# Autodesk Inventor assembly: Catapult Launcher
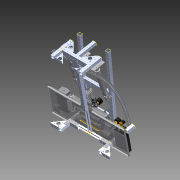
[picture p0: Inventor's stored thumbnail of the model, 180x180]
Saved by Autodesk Inventor 2014 SP1 (Build 180222100, 222)
## iProperties
Created: 2014-01-17
Part Number: Catapult Launcher
Document SubType Name: Assembly
Designer: Andrew Toennies
Mass: 5501.43 g
Surface Area: 13469.8 cm^2
Volume: 1150.51 cm^3
Density: 4.78173 g/cm^3
Author: Andrew Toennies
## Documents named in this file (38)
- C:\Users\Arpan\Documents\GitHub\2014buildCAD\New Shooter\Catapult Launcher.iam
- C:\Users\Arpan\Documents\GitHub\2014buildCAD\New Shooter\Vex Pro Side Bearing Gusset - OUT OF STOCK 1192014.ipt
- C:\Users\Arpan\Documents\GitHub\2014buildCAD\New Shooter\Vex Pro Corner Gusset - IN STOCK 1192014.ipt
- C:\Users\Arpan\Documents\GitHub\2014buildCAD\New Shooter\Bearing ID 0.500 Hex OD 1.125.ipt
- C:\Users\Arpan\Documents\GitHub\2014buildCAD\New Shooter\Shaft (Steel 0.500 Hex).ipt
- C:\Users\Arpan\Documents\GitHub\2014buildCAD\New Shooter\1.5 in bore 6 in stroke cylinder - BIMBA\176-DP(D-229)(F,D-231-1).iam
- C:\Users\Arpan\Documents\GitHub\2014buildCAD\New Shooter\Aluminum Plate (0.125).ipt
- C:\Users\Arpan\Documents\GitHub\2014buildCAD\New Shooter\1.5 in bore 6 in stroke cylinder - BIMBA\D-14826.ipt
- C:\Users\Arpan\Documents\GitHub\2014buildCAD\New Shooter\1.5 in bore 6 in stroke cylinder - BIMBA\D-9969.ipt
- C:\Users\Arpan\Documents\GitHub\2014buildCAD\New Shooter\Vex Pro End Bearing Mount - IN STOCK 1192014.ipt
- C:\Users\Arpan\Documents\GitHub\2014buildCAD\New Shooter\Vex Pro 1x1 rectangular tubing 13 in length.ipt
- C:\Users\Arpan\Documents\GitHub\2014buildCAD\New Shooter\Vex Pro 1x1 rectangular tubing 25 in length.ipt
- C:\Users\Arpan\Documents\GitHub\2014buildCAD\New Shooter\0.5625 in bore 2 in stroke compact cylinder - BIMBA\FO-022.iam
- C:\Users\Arpan\Documents\GitHub\2014buildCAD\New Shooter\Hex Shaft Collar 1-2 in (7552K500).ipt
- C:\Users\Arpan\Documents\GitHub\2014buildCAD\New Shooter\#8 1 in length standoff 93330A459.ipt
- C:\Users\Arpan\Documents\GitHub\2014buildCAD\New Shooter\Ramp.ipt
- C:\Users\Arpan\Documents\GitHub\2014buildCAD\New folder (2)\Pneumatics_Clippard_AVT-32-16.iam
- C:\Users\Arpan\Documents\GitHub\2014buildCAD\New Shooter\Vex Pro T gusset - OUT OF STOCK 1192014.ipt
- C:\Users\Arpan\Documents\GitHub\2014buildCAD\New Shooter\#8 0.250 in length spacer 92510A462.ipt
- C:\Users\Arpan\Documents\GitHub\2014buildCAD\New Shooter\#8 0.625 in length spacer 92510A466.ipt
- C:\Users\Arpan\Documents\GitHub\2014buildCAD\New Shooter\Vex Pro 1x1 rectangular tubing 12 in length.ipt
- C:\Users\Arpan\Documents\GitHub\2014buildCAD\New Shooter\Vex Pro 1x1 rectangular tubing 24.5 in length.ipt
- C:\Users\Arpan\Documents\GitHub\2014buildCAD\New Shooter\Vex Pro 1x1 rectangular tubing 7 in length.ipt
- C:\Users\Arpan\Documents\GitHub\2014buildCAD\New Shooter\Vex Pro 1x1 rectangular tubing 9 in length.ipt
- C:\Users\Arpan\Documents\GitHub\2014buildCAD\New Shooter\Vex Pro 1x1 rectangular tubing 6.125 in length.ipt
- C:\Users\Arpan\Documents\GitHub\2014buildCAD\New Shooter\Spacer (0.630 in ID 1 in OD) aluminum.ipt
- C:\Users\Arpan\Documents\GitHub\2014buildCAD\big air tank\Pneumatics_Clippard_AVT-32-32.iam
- C:\Users\Arpan\Documents\GitHub\2014buildCAD\pneumatics board\pneumatics thing 2.iam
- C:\Users\Arpan\Documents\GitHub\2014buildCAD\New Shooter\Manifold and Valves\Manifold.iam
- C:\Users\Arpan\Documents\GitHub\2014buildCAD\pneumatics board\pneumatic thing 1.iam
- C:\Users\Arpan\Documents\GitHub\2014buildCAD\electrical\CS_Converter_CLL25-24S05.ipt
- C:\Users\Arpan\Documents\GitHub\2014buildCAD\electrical\CS_WirelessBridge_DAP1522.ipt
- C:\Users\Arpan\Documents\GitHub\2014buildCAD\New Shooter\Pneumatics Board.ipt
- C:\Users\Arpan\Documents\GitHub\2014buildCAD\New Shooter\Aluminum Angle 2.ipt
- C:\Users\Arpan\Documents\GitHub\2014buildCAD\New Shooter\Aluminum Angle 1 Left.ipt
- C:\Users\Arpan\Documents\GitHub\2014buildCAD\New Shooter\Aluminum Angle 1 Right.ipt
- C:\Users\Arpan\Documents\GitHub\2014buildCAD\New Shooter\Aluminum Angle 3 Left.ipt
- C:\Users\Arpan\Documents\GitHub\2014buildCAD\New Shooter\Aluminum Angle 3 Right.ipt
## Components (98 placed, 37 different names)
1. Vex Pro T gusset - OUT OF STOCK 1192014:2 — Mate:376, Flush:71, Flush:72
2. Vex Pro T gusset - OUT OF STOCK 1192014:1 — Mate:375, Flush:69, Flush:70
3. #8 1 in length standoff 93330A459:12 — Mate:342, Mate:343
4. #8 1 in length standoff 93330A459:11 — Mate:340, Mate:341
5. #8 1 in length standoff 93330A459:10 — Mate:338, Mate:339
6. #8 1 in length standoff 93330A459:9 — Mate:336, Mate:337
7. #8 1 in length standoff 93330A459:6 — Mate:325, Mate:326
8. #8 1 in length standoff 93330A459:1 — Mate:319, Mate:320
9. #8 1 in length standoff 93330A459:2 — Mate:321, Mate:322
10. #8 1 in length standoff 93330A459:5 — Mate:323, Mate:324
11. Vex Pro 1x1 rectangular tubing 12 in length:1 — Flush:1, Flush:2, Mate:8, Mate:11, Mate:195, Flush:32, Flush:33, Flush:34, Flush:35, Mate:278, Flush:51, Mate:352, Mate:376, Flush:71, Mate:380, Mate:381, Mate:390, Flush:77, Flush:78, Mate:403, Mate:405
12. Vex Pro 1x1 rectangular tubing 12 in length:2 — Flush:1, Flush:2, Mate:3, Mate:5, Mate:123, Mate:188, Mate:195, Flush:25, Flush:28, Flush:29, Flush:30, Flush:31, Mate:355, Mate:375, Flush:69, Mate:378, Mate:389, Flush:75, Flush:76
13. Vex Pro Side Bearing Gusset - OUT OF STOCK 1192014:1 — Mate:3, Mate:26, Mate:27, Flush:28, Flush:29, Mate:319, Mate:320, Mate:322, Mate:324, Mate:326
14. Vex Pro Side Bearing Gusset - OUT OF STOCK 1192014:2 — Mate:5, Mate:28, Mate:29, Flush:30, Flush:31, Mate:321, Mate:323, Mate:325
15. Vex Pro Side Bearing Gusset - OUT OF STOCK 1192014:3 — Mate:11, Mate:32, Mate:33, Flush:32, Flush:33, Mate:337, Mate:338, Mate:339, Mate:340, Mate:342, Mate:343
16. Vex Pro Side Bearing Gusset - OUT OF STOCK 1192014:4 — Mate:8, Mate:30, Mate:31, Flush:34, Flush:35, Mate:336, Mate:341
17. Vex Pro Corner Gusset - IN STOCK 1192014:2 — Mate:389, Flush:75, Flush:76
18. Vex Pro Corner Gusset - IN STOCK 1192014:4 — Mate:390, Flush:77, Flush:78
19. Bearing ID 0.500 Hex OD 1.125:1 — Mate:28, Mate:29, Flush:3, Flush:5, Mate:306
20. Bearing ID 0.500 Hex OD 1.125:2 — Mate:26, Mate:27, Flush:3, Mate:34, Mate:35, Mate:303
21. Bearing ID 0.500 Hex OD 1.125:3 — Mate:30, Mate:31, Flush:4, Mate:318
22. Bearing ID 0.500 Hex OD 1.125:4 — Mate:32, Mate:33, Flush:4, Flush:5, Mate:69, Mate:315
23. Pneumatics_Clippard_AVT-32-16:1 [sub-assembly] — Tangent:8, Flush:94, Tangent:11, Tangent:12
24. Pneumatics_Clippard_AVT-32-16:2 [sub-assembly] — Tangent:10, Flush:94, Tangent:11, Tangent:13, Flush:101
25. Pneumatics_Clippard_AVT-32-32:1 [sub-assembly] — Mate:403, Tangent:2, Flush:87, Tangent:9, Tangent:12
26. Pneumatics_Clippard_AVT-32-32:2 [sub-assembly] — Flush:87, Tangent:7, Tangent:13, Flush:101
27. Manifold:1 [sub-assembly] — Mate:406, Flush:97, Flush:98
28. pneumatic thing 1:1 [sub-assembly] — Mate:408, Flush:92, Flush:93
29. CS_Converter_CLL25-24S05:1 — Mate:410, Mate:414, Mate:415
30. CS_WirelessBridge_DAP1522:1 — Mate:409, Flush:90, Flush:91
31. Pneumatics Board:1 — Mate:404, Mate:405, Flush:89, Mate:406, Mate:408, Mate:409, Mate:410, Flush:90, Flush:91, Flush:92, Flush:93, Tangent:7, Tangent:8, Tangent:9, Tangent:10, Mate:413, Flush:97, Mate:414, Mate:415, Flush:98, Flush:99, Flush:100, Mate:418, Flush:102, Mate:419, Mate:420, Flush:103, Mate:421, Flush:104, Mate:422, Mate:423, Mate:424, Mate:425, Flush:105, Mate:426, Flush:106, Mate:428, Flush:107
32. pneumatics thing 2:2 [sub-assembly] — Mate:413, Flush:99, Flush:100
33. #8 1 in length standoff 93330A459:13 — Mate:350, Mate:351
34. #8 1 in length standoff 93330A459:14 — Mate:348, Mate:349
35. #8 1 in length standoff 93330A459:15 — Mate:346, Mate:347
36. #8 1 in length standoff 93330A459:16 — Mate:344, Mate:345
37. #8 1 in length standoff 93330A459:3 — Mate:327, Mate:328
38. #8 1 in length standoff 93330A459:4 — Mate:329, Mate:330
39. #8 1 in length standoff 93330A459:7 — Mate:334, Mate:335
40. #8 1 in length standoff 93330A459:8 — Mate:332, Mate:333
41. Vex Pro Corner Gusset - IN STOCK 1192014:14 — Mate:250, Mate:251, Flush:45, Mate:271
42. Vex Pro Corner Gusset - IN STOCK 1192014:13 — Mate:252, Mate:253, Flush:46
43. Vex Pro Corner Gusset - IN STOCK 1192014:12 — Mate:248, Mate:249, Flush:44
44. Vex Pro Corner Gusset - IN STOCK 1192014:11 — Mate:243, Flush:43, Mate:244
45. Vex Pro 1x1 rectangular tubing 9 in length:1 — Mate:191, Flush:42, Mate:250, Mate:253, Flush:46, Mate:267
46. Vex Pro 1x1 rectangular tubing 9 in length:2 — Flush:41, Mate:242, Mate:243, Flush:43, Mate:246, Mate:248, Flush:44
47. D-9969:1 — Mate:164, Mate:165, Mate:198, Flush:36, Mate:270, Mate:377
48. D-14826:1 — Mate:164, Mate:169, Mate:170, Flush:37, Mate:247
49. Vex Pro End Bearing Mount - IN STOCK 1192014:4 — Mate:229, Mate:230, Mate:231, Mate:232, Mate:246, Mate:345, Mate:346, Mate:348, Mate:349, Mate:350
50. Vex Pro End Bearing Mount - IN STOCK 1192014:3 — Mate:217, Mate:218, Mate:219, Mate:220, Mate:221, Mate:327, Mate:328, Mate:330, Mate:333, Mate:335
51. Vex Pro End Bearing Mount - IN STOCK 1192014:2 — Mate:233, Mate:234, Mate:235, Mate:236, Mate:245, Mate:344, Mate:347, Mate:351
52. Vex Pro End Bearing Mount - IN STOCK 1192014:1 — Mate:222, Mate:223, Mate:224, Mate:225, Mate:226, Mate:329, Mate:332, Mate:334
53. Vex Pro 1x1 rectangular tubing 24.5 in length:2 — Mate:198, Mate:229, Mate:230, Mate:231, Mate:233, Mate:234, Mate:235, Flush:27, Flush:36, Flush:41, Mate:242, Mate:244, Mate:251, Flush:45, Mate:267, Mate:270, Mate:271
54. Vex Pro 1x1 rectangular tubing 24.5 in length:1 — Mate:188, Mate:191, Mate:212, Mate:219, Mate:220, Mate:221, Mate:224, Mate:225, Mate:226, Flush:26, Flush:37, Flush:42, Mate:247, Mate:249, Mate:252
55. Bearing ID 0.500 Hex OD 1.125:5 — Mate:80, Mate:222, Mate:223, Mate:228, Mate:309
56. Bearing ID 0.500 Hex OD 1.125:6 — Mate:80, Mate:217, Mate:218, Mate:227
57. Bearing ID 0.500 Hex OD 1.125:7 — Mate:68, Mate:69, Mate:236, Mate:245, Mate:397
58. Bearing ID 0.500 Hex OD 1.125:8 — Mate:68, Mate:232, Mate:312
59. Vex Pro T gusset - OUT OF STOCK 1192014:3 — Mate:388, Flush:73, Flush:74
60. Aluminum Plate (0.125):1 — Mate:153, Mate:159, Mate:434, Mate:435, Mate:436, Mate:437
61. Aluminum Plate (0.125):2 — Mate:156, Mate:160, Mate:430, Mate:431, Mate:432, Mate:433
62. Vex Pro 1x1 rectangular tubing 7 in length:2 — Flush:19, Mate:159, Flush:27, Mate:276, Mate:359, Mate:385, Mate:391, Flush:79, Flush:80, Mate:430, Mate:431
63. Vex Pro 1x1 rectangular tubing 7 in length:1 — Mate:123, Flush:19, Mate:160, Mate:212, Flush:26, Mate:272, Flush:48, Mate:273, Mate:275, Mate:360, Mate:387, Mate:392, Flush:81, Flush:82, Mate:434, Mate:435
64. Vex Pro Corner Gusset - IN STOCK 1192014:8 — Mate:392, Flush:81, Flush:82
65. Vex Pro Corner Gusset - IN STOCK 1192014:6 — Mate:391, Flush:79, Flush:80
66. Vex Pro 1x1 rectangular tubing 9 in length:3 — Mate:272, Flush:48, Mate:274, Flush:49, Mate:277, Flush:50, Mate:290, Mate:291, Mate:293, Flush:57, Mate:369, Flush:66
67. Vex Pro Corner Gusset - IN STOCK 1192014:15 — Mate:273, Mate:274, Flush:49, Mate:275
68. Vex Pro Corner Gusset - IN STOCK 1192014:16 — Mate:276, Mate:277, Flush:50
69. Vex Pro 1x1 rectangular tubing 13 in length:1 — Mate:278, Flush:51, Mate:284, Flush:55, Flush:70, Flush:72, Mate:388, Flush:73, Tangent:2, Mate:404, Flush:89
70. Vex Pro 1x1 rectangular tubing 25 in length:1 — Mate:284, Flush:55, Mate:285, Mate:289, Flush:56, Mate:292, Mate:300, Flush:67, Flush:74, Mate:416, Mate:417
71. FO-022:1 [sub-assembly] — Mate:285, Mate:416, Mate:417
72. Vex Pro Corner Gusset - IN STOCK 1192014:17 — Mate:289, Mate:290, Flush:56, Mate:291
73. Vex Pro Corner Gusset - IN STOCK 1192014:18 — Mate:292, Mate:293, Flush:57
74. Vex Pro 1x1 rectangular tubing 6.125 in length:1 — Mate:369, Flush:66, Mate:370, Flush:68
75. Vex Pro Corner Gusset - IN STOCK 1192014:21 — Mate:300, Mate:370, Flush:67, Flush:68
76. #8 0.250 in length spacer 92510A462:1 — Mate:380, Mate:381, Mate:382
77. #8 0.250 in length spacer 92510A462:2 — Mate:378, Mate:379, Mate:383
78. #8 0.625 in length spacer 92510A466:1 — Mate:384, Mate:385
79. #8 0.625 in length spacer 92510A466:2 — Mate:386, Mate:387
80. Ramp:1 — Mate:355, Mate:360, Mate:379, Mate:383, Mate:386
81. Ramp:2 — Mate:352, Mate:359, Mate:382, Mate:384
82. Aluminum Angle 2:1 — Mate:418, Flush:102, Mate:419, Mate:429
83. Aluminum Angle 2:2 — Mate:420, Flush:103, Mate:421, Mate:427
84. Aluminum Angle 1 Left:1 — Flush:104, Mate:422, Mate:423
85. Aluminum Angle 1 Right:1 — Mate:424, Mate:425, Flush:105
86. Aluminum Angle 3 Left:1 — Mate:426, Flush:106, Mate:427
87. Aluminum Angle 3 Right:1 — Mate:428, Mate:429, Flush:107
88. Spacer (0.630 in ID 1 in OD) aluminum:1 — Mate:399, Mate:400
89. Spacer (0.630 in ID 1 in OD) aluminum:2 — Mate:397, Mate:398
90. Shaft (Steel 0.500 Hex):1 — Mate:34, Mate:35, Flush:25, Mate:227, Mate:228, Mate:301, Mate:302, Mate:304, Mate:305, Mate:307, Mate:308, Mate:310, Mate:311, Mate:313, Mate:314, Mate:316, Mate:317
91. Hex Shaft Collar 1-2 in (7552K500):1 — Mate:301, Mate:302, Mate:303
92. Hex Shaft Collar 1-2 in (7552K500):2 — Mate:307, Mate:308, Mate:309
93. Hex Shaft Collar 1-2 in (7552K500):3 — Mate:304, Mate:305, Mate:306, Mate:399, Mate:400
94. Hex Shaft Collar 1-2 in (7552K500):4 — Mate:310, Mate:311, Mate:312
95. Hex Shaft Collar 1-2 in (7552K500):5 — Mate:313, Mate:314, Mate:315, Mate:398
96. Hex Shaft Collar 1-2 in (7552K500):6 — Mate:316, Mate:317, Mate:318
97. 176-DP(D-229)(F,D-231-1):1 [sub-assembly] — Mate:153, Mate:165, Mate:171, Mate:377, Mate:432, Mate:433
98. 176-DP(D-229)(F,D-231-1):2 [sub-assembly] — Mate:156, Mate:169, Mate:170, Mate:171, Mate:436, Mate:437
## Relationships (267: Mate 192, Flush 67, Tangent 8)
- Flush:1: Vex Pro 1x1 rectangular tubing 12 in length:1 ↔ Vex Pro 1x1 rectangular tubing 12 in length:2
- Flush:2: Vex Pro 1x1 rectangular tubing 12 in length:1 ↔ Vex Pro 1x1 rectangular tubing 12 in length:2
- Mate:3: Vex Pro 1x1 rectangular tubing 12 in length:2 ↔ Vex Pro Side Bearing Gusset - OUT OF STOCK 1192014:1
- Mate:5: Vex Pro 1x1 rectangular tubing 12 in length:2 ↔ Vex Pro Side Bearing Gusset - OUT OF STOCK 1192014:2
- Mate:8: Vex Pro 1x1 rectangular tubing 12 in length:1 ↔ Vex Pro Side Bearing Gusset - OUT OF STOCK 1192014:4
- Mate:11: Vex Pro 1x1 rectangular tubing 12 in length:1 ↔ Vex Pro Side Bearing Gusset - OUT OF STOCK 1192014:3
- Mate:26: Vex Pro Side Bearing Gusset - OUT OF STOCK 1192014:1 ↔ Bearing ID 0.500 Hex OD 1.125:2
- Mate:27: Vex Pro Side Bearing Gusset - OUT OF STOCK 1192014:1 ↔ Bearing ID 0.500 Hex OD 1.125:2
- Mate:28: Vex Pro Side Bearing Gusset - OUT OF STOCK 1192014:2 ↔ Bearing ID 0.500 Hex OD 1.125:1
- Mate:29: Vex Pro Side Bearing Gusset - OUT OF STOCK 1192014:2 ↔ Bearing ID 0.500 Hex OD 1.125:1
- Flush:3: Bearing ID 0.500 Hex OD 1.125:1 ↔ Bearing ID 0.500 Hex OD 1.125:2
- Mate:30: Vex Pro Side Bearing Gusset - OUT OF STOCK 1192014:4 ↔ Bearing ID 0.500 Hex OD 1.125:3
- Mate:31: Vex Pro Side Bearing Gusset - OUT OF STOCK 1192014:4 ↔ Bearing ID 0.500 Hex OD 1.125:3
- Mate:32: Vex Pro Side Bearing Gusset - OUT OF STOCK 1192014:3 ↔ Bearing ID 0.500 Hex OD 1.125:4
- Mate:33: Vex Pro Side Bearing Gusset - OUT OF STOCK 1192014:3 ↔ Bearing ID 0.500 Hex OD 1.125:4
- Flush:4: Bearing ID 0.500 Hex OD 1.125:3 ↔ Bearing ID 0.500 Hex OD 1.125:4
- Flush:5: Bearing ID 0.500 Hex OD 1.125:1 ↔ Bearing ID 0.500 Hex OD 1.125:4
- Mate:34: Bearing ID 0.500 Hex OD 1.125:2 ↔ Shaft (Steel 0.500 Hex):1
- Mate:35: Bearing ID 0.500 Hex OD 1.125:2 ↔ Shaft (Steel 0.500 Hex):1
- Mate:68: Bearing ID 0.500 Hex OD 1.125:7 ↔ Bearing ID 0.500 Hex OD 1.125:8
- Mate:69: Bearing ID 0.500 Hex OD 1.125:4 ↔ Bearing ID 0.500 Hex OD 1.125:7
- Mate:80: Bearing ID 0.500 Hex OD 1.125:5 ↔ Bearing ID 0.500 Hex OD 1.125:6
- Mate:123 (-685.8 mm): Vex Pro 1x1 rectangular tubing 12 in length:2 ↔ Vex Pro 1x1 rectangular tubing 7 in length:1
- Flush:19: Vex Pro 1x1 rectangular tubing 7 in length:2 ↔ Vex Pro 1x1 rectangular tubing 7 in length:1
- Mate:153: Aluminum Plate (0.125):1 ↔ 176-DP(D-229)(F,D-231-1):1
- Mate:156: Aluminum Plate (0.125):2 ↔ 176-DP(D-229)(F,D-231-1):2
- Mate:159: Aluminum Plate (0.125):1 ↔ Vex Pro 1x1 rectangular tubing 7 in length:2
- Mate:160: Aluminum Plate (0.125):2 ↔ Vex Pro 1x1 rectangular tubing 7 in length:1
- Mate:164: D-9969:1 ↔ D-14826:1
- Mate:165: D-9969:1 ↔ 176-DP(D-229)(F,D-231-1):1
- Mate:169: D-14826:1 ↔ 176-DP(D-229)(F,D-231-1):2
- Mate:170: D-14826:1 ↔ 176-DP(D-229)(F,D-231-1):2
- Mate:171: 176-DP(D-229)(F,D-231-1):1 ↔ 176-DP(D-229)(F,D-231-1):2
- Mate:188 (25.4 mm): Vex Pro 1x1 rectangular tubing 12 in length:2 ↔ Vex Pro 1x1 rectangular tubing 24.5 in length:1
- Mate:191: Vex Pro 1x1 rectangular tubing 9 in length:1 ↔ Vex Pro 1x1 rectangular tubing 24.5 in length:1
- Mate:195 (330.2 mm): Vex Pro 1x1 rectangular tubing 12 in length:1 ↔ Vex Pro 1x1 rectangular tubing 12 in length:2
- Flush:25 (-25.4 mm): Vex Pro 1x1 rectangular tubing 12 in length:2 ↔ Shaft (Steel 0.500 Hex):1
- Mate:198: D-9969:1 ↔ Vex Pro 1x1 rectangular tubing 24.5 in length:2
- Mate:212: Vex Pro 1x1 rectangular tubing 24.5 in length:1 ↔ Vex Pro 1x1 rectangular tubing 7 in length:1
- Mate:217: Vex Pro End Bearing Mount - IN STOCK 1192014:3 ↔ Bearing ID 0.500 Hex OD 1.125:6
- Mate:218: Vex Pro End Bearing Mount - IN STOCK 1192014:3 ↔ Bearing ID 0.500 Hex OD 1.125:6
- Mate:219: Vex Pro End Bearing Mount - IN STOCK 1192014:3 ↔ Vex Pro 1x1 rectangular tubing 24.5 in length:1
- Mate:220: Vex Pro End Bearing Mount - IN STOCK 1192014:3 ↔ Vex Pro 1x1 rectangular tubing 24.5 in length:1
- Mate:221: Vex Pro End Bearing Mount - IN STOCK 1192014:3 ↔ Vex Pro 1x1 rectangular tubing 24.5 in length:1
- Mate:222: Vex Pro End Bearing Mount - IN STOCK 1192014:1 ↔ Bearing ID 0.500 Hex OD 1.125:5
- Mate:223: Vex Pro End Bearing Mount - IN STOCK 1192014:1 ↔ Bearing ID 0.500 Hex OD 1.125:5
- Mate:224: Vex Pro End Bearing Mount - IN STOCK 1192014:1 ↔ Vex Pro 1x1 rectangular tubing 24.5 in length:1
- Mate:225: Vex Pro End Bearing Mount - IN STOCK 1192014:1 ↔ Vex Pro 1x1 rectangular tubing 24.5 in length:1
- Mate:226: Vex Pro End Bearing Mount - IN STOCK 1192014:1 ↔ Vex Pro 1x1 rectangular tubing 24.5 in length:1
- Mate:227: Bearing ID 0.500 Hex OD 1.125:6 ↔ Shaft (Steel 0.500 Hex):1
- Mate:228: Bearing ID 0.500 Hex OD 1.125:5 ↔ Shaft (Steel 0.500 Hex):1
- Mate:229: Vex Pro End Bearing Mount - IN STOCK 1192014:4 ↔ Vex Pro 1x1 rectangular tubing 24.5 in length:2
- Mate:230: Vex Pro End Bearing Mount - IN STOCK 1192014:4 ↔ Vex Pro 1x1 rectangular tubing 24.5 in length:2
- Mate:231: Vex Pro End Bearing Mount - IN STOCK 1192014:4 ↔ Vex Pro 1x1 rectangular tubing 24.5 in length:2
- Mate:232: Vex Pro End Bearing Mount - IN STOCK 1192014:4 ↔ Bearing ID 0.500 Hex OD 1.125:8
- Mate:233: Vex Pro End Bearing Mount - IN STOCK 1192014:2 ↔ Vex Pro 1x1 rectangular tubing 24.5 in length:2
- Mate:234: Vex Pro End Bearing Mount - IN STOCK 1192014:2 ↔ Vex Pro 1x1 rectangular tubing 24.5 in length:2
- Mate:235: Vex Pro End Bearing Mount - IN STOCK 1192014:2 ↔ Vex Pro 1x1 rectangular tubing 24.5 in length:2
- Mate:236: Vex Pro End Bearing Mount - IN STOCK 1192014:2 ↔ Bearing ID 0.500 Hex OD 1.125:7
- Flush:26: Vex Pro 1x1 rectangular tubing 24.5 in length:1 ↔ Vex Pro 1x1 rectangular tubing 7 in length:1
- Flush:27: Vex Pro 1x1 rectangular tubing 24.5 in length:2 ↔ Vex Pro 1x1 rectangular tubing 7 in length:2
- Flush:28: Vex Pro 1x1 rectangular tubing 12 in length:2 ↔ Vex Pro Side Bearing Gusset - OUT OF STOCK 1192014:1
- Flush:29 (82.55 mm): Vex Pro 1x1 rectangular tubing 12 in length:2 ↔ Vex Pro Side Bearing Gusset - OUT OF STOCK 1192014:1
- Flush:30: Vex Pro 1x1 rectangular tubing 12 in length:2 ↔ Vex Pro Side Bearing Gusset - OUT OF STOCK 1192014:2
- Flush:31 (-82.55 mm): Vex Pro 1x1 rectangular tubing 12 in length:2 ↔ Vex Pro Side Bearing Gusset - OUT OF STOCK 1192014:2
- Flush:32: Vex Pro 1x1 rectangular tubing 12 in length:1 ↔ Vex Pro Side Bearing Gusset - OUT OF STOCK 1192014:3
- Flush:33 (82.55 mm): Vex Pro 1x1 rectangular tubing 12 in length:1 ↔ Vex Pro Side Bearing Gusset - OUT OF STOCK 1192014:3
- Flush:34: Vex Pro 1x1 rectangular tubing 12 in length:1 ↔ Vex Pro Side Bearing Gusset - OUT OF STOCK 1192014:4
- Flush:35 (-82.55 mm): Vex Pro 1x1 rectangular tubing 12 in length:1 ↔ Vex Pro Side Bearing Gusset - OUT OF STOCK 1192014:4
- Flush:36: D-9969:1 ↔ Vex Pro 1x1 rectangular tubing 24.5 in length:2
- Flush:37: D-14826:1 ↔ Vex Pro 1x1 rectangular tubing 24.5 in length:1
- Flush:41: Vex Pro 1x1 rectangular tubing 9 in length:2 ↔ Vex Pro 1x1 rectangular tubing 24.5 in length:2
- Mate:242: Vex Pro 1x1 rectangular tubing 9 in length:2 ↔ Vex Pro 1x1 rectangular tubing 24.5 in length:2
- Flush:42: Vex Pro 1x1 rectangular tubing 9 in length:1 ↔ Vex Pro 1x1 rectangular tubing 24.5 in length:1
- Mate:243: Vex Pro Corner Gusset - IN STOCK 1192014:11 ↔ Vex Pro 1x1 rectangular tubing 9 in length:2
- Flush:43: Vex Pro Corner Gusset - IN STOCK 1192014:11 ↔ Vex Pro 1x1 rectangular tubing 9 in length:2
- Mate:244: Vex Pro Corner Gusset - IN STOCK 1192014:11 ↔ Vex Pro 1x1 rectangular tubing 24.5 in length:2
- Mate:245: Vex Pro End Bearing Mount - IN STOCK 1192014:2 ↔ Bearing ID 0.500 Hex OD 1.125:7
- Mate:246 (6.35 mm): Vex Pro 1x1 rectangular tubing 9 in length:2 ↔ Vex Pro End Bearing Mount - IN STOCK 1192014:4
- Mate:247: D-14826:1 ↔ Vex Pro 1x1 rectangular tubing 24.5 in length:1
- Mate:248: Vex Pro Corner Gusset - IN STOCK 1192014:12 ↔ Vex Pro 1x1 rectangular tubing 9 in length:2
- Mate:249: Vex Pro Corner Gusset - IN STOCK 1192014:12 ↔ Vex Pro 1x1 rectangular tubing 24.5 in length:1
- Flush:44: Vex Pro Corner Gusset - IN STOCK 1192014:12 ↔ Vex Pro 1x1 rectangular tubing 9 in length:2
- Mate:250: Vex Pro Corner Gusset - IN STOCK 1192014:14 ↔ Vex Pro 1x1 rectangular tubing 9 in length:1
- Mate:251: Vex Pro Corner Gusset - IN STOCK 1192014:14 ↔ Vex Pro 1x1 rectangular tubing 24.5 in length:2
- Flush:45: Vex Pro Corner Gusset - IN STOCK 1192014:14 ↔ Vex Pro 1x1 rectangular tubing 24.5 in length:2
- Mate:252: Vex Pro Corner Gusset - IN STOCK 1192014:13 ↔ Vex Pro 1x1 rectangular tubing 24.5 in length:1
- Mate:253: Vex Pro Corner Gusset - IN STOCK 1192014:13 ↔ Vex Pro 1x1 rectangular tubing 9 in length:1
- Flush:46: Vex Pro Corner Gusset - IN STOCK 1192014:13 ↔ Vex Pro 1x1 rectangular tubing 9 in length:1
- Mate:267: Vex Pro 1x1 rectangular tubing 9 in length:1 ↔ Vex Pro 1x1 rectangular tubing 24.5 in length:2
- Mate:270: D-9969:1 ↔ Vex Pro 1x1 rectangular tubing 24.5 in length:2
- Mate:271: Vex Pro Corner Gusset - IN STOCK 1192014:14 ↔ Vex Pro 1x1 rectangular tubing 24.5 in length:2
- Mate:272: Vex Pro 1x1 rectangular tubing 7 in length:1 ↔ Vex Pro 1x1 rectangular tubing 9 in length:3
- Flush:48: Vex Pro 1x1 rectangular tubing 7 in length:1 ↔ Vex Pro 1x1 rectangular tubing 9 in length:3
- Mate:273: Vex Pro 1x1 rectangular tubing 7 in length:1 ↔ Vex Pro Corner Gusset - IN STOCK 1192014:15
- Mate:274: Vex Pro 1x1 rectangular tubing 9 in length:3 ↔ Vex Pro Corner Gusset - IN STOCK 1192014:15
- Flush:49: Vex Pro 1x1 rectangular tubing 9 in length:3 ↔ Vex Pro Corner Gusset - IN STOCK 1192014:15
- Mate:275: Vex Pro 1x1 rectangular tubing 7 in length:1 ↔ Vex Pro Corner Gusset - IN STOCK 1192014:15
- Mate:276: Vex Pro 1x1 rectangular tubing 7 in length:2 ↔ Vex Pro Corner Gusset - IN STOCK 1192014:16
- Mate:277: Vex Pro 1x1 rectangular tubing 9 in length:3 ↔ Vex Pro Corner Gusset - IN STOCK 1192014:16
- Flush:50: Vex Pro 1x1 rectangular tubing 9 in length:3 ↔ Vex Pro Corner Gusset - IN STOCK 1192014:16
- Mate:278: Vex Pro 1x1 rectangular tubing 12 in length:1 ↔ Vex Pro 1x1 rectangular tubing 13 in length:1
- Flush:51: Vex Pro 1x1 rectangular tubing 12 in length:1 ↔ Vex Pro 1x1 rectangular tubing 13 in length:1
- Mate:284: Vex Pro 1x1 rectangular tubing 13 in length:1 ↔ Vex Pro 1x1 rectangular tubing 25 in length:1
- Flush:55: Vex Pro 1x1 rectangular tubing 13 in length:1 ↔ Vex Pro 1x1 rectangular tubing 25 in length:1
- Mate:285: Vex Pro 1x1 rectangular tubing 25 in length:1 ↔ FO-022:1
- Mate:289: Vex Pro 1x1 rectangular tubing 25 in length:1 ↔ Vex Pro Corner Gusset - IN STOCK 1192014:17
- Mate:290: Vex Pro 1x1 rectangular tubing 9 in length:3 ↔ Vex Pro Corner Gusset - IN STOCK 1192014:17
- Flush:56: Vex Pro 1x1 rectangular tubing 25 in length:1 ↔ Vex Pro Corner Gusset - IN STOCK 1192014:17
- Mate:291: Vex Pro 1x1 rectangular tubing 9 in length:3 ↔ Vex Pro Corner Gusset - IN STOCK 1192014:17
- Mate:292: Vex Pro 1x1 rectangular tubing 25 in length:1 ↔ Vex Pro Corner Gusset - IN STOCK 1192014:18
- Mate:293: Vex Pro 1x1 rectangular tubing 9 in length:3 ↔ Vex Pro Corner Gusset - IN STOCK 1192014:18
- Flush:57: Vex Pro 1x1 rectangular tubing 9 in length:3 ↔ Vex Pro Corner Gusset - IN STOCK 1192014:18
- Mate:300: Vex Pro 1x1 rectangular tubing 25 in length:1 ↔ Vex Pro Corner Gusset - IN STOCK 1192014:21
- Mate:301: Shaft (Steel 0.500 Hex):1 ↔ Hex Shaft Collar 1-2 in (7552K500):1
- Mate:302: Shaft (Steel 0.500 Hex):1 ↔ Hex Shaft Collar 1-2 in (7552K500):1
- Mate:303: Bearing ID 0.500 Hex OD 1.125:2 ↔ Hex Shaft Collar 1-2 in (7552K500):1
- Mate:304: Shaft (Steel 0.500 Hex):1 ↔ Hex Shaft Collar 1-2 in (7552K500):3
- Mate:305: Shaft (Steel 0.500 Hex):1 ↔ Hex Shaft Collar 1-2 in (7552K500):3
- Mate:306: Bearing ID 0.500 Hex OD 1.125:1 ↔ Hex Shaft Collar 1-2 in (7552K500):3
- Mate:307: Shaft (Steel 0.500 Hex):1 ↔ Hex Shaft Collar 1-2 in (7552K500):2
- Mate:308: Shaft (Steel 0.500 Hex):1 ↔ Hex Shaft Collar 1-2 in (7552K500):2
- Mate:309: Bearing ID 0.500 Hex OD 1.125:5 ↔ Hex Shaft Collar 1-2 in (7552K500):2
- Mate:310: Shaft (Steel 0.500 Hex):1 ↔ Hex Shaft Collar 1-2 in (7552K500):4
- Mate:311: Shaft (Steel 0.500 Hex):1 ↔ Hex Shaft Collar 1-2 in (7552K500):4
- Mate:312: Bearing ID 0.500 Hex OD 1.125:8 ↔ Hex Shaft Collar 1-2 in (7552K500):4
- Mate:313: Shaft (Steel 0.500 Hex):1 ↔ Hex Shaft Collar 1-2 in (7552K500):5
- Mate:314: Shaft (Steel 0.500 Hex):1 ↔ Hex Shaft Collar 1-2 in (7552K500):5
- Mate:315: Bearing ID 0.500 Hex OD 1.125:4 ↔ Hex Shaft Collar 1-2 in (7552K500):5
- Mate:316: Shaft (Steel 0.500 Hex):1 ↔ Hex Shaft Collar 1-2 in (7552K500):6
- Mate:317: Shaft (Steel 0.500 Hex):1 ↔ Hex Shaft Collar 1-2 in (7552K500):6
- Mate:318: Bearing ID 0.500 Hex OD 1.125:3 ↔ Hex Shaft Collar 1-2 in (7552K500):6
- Mate:319: #8 1 in length standoff 93330A459:1 ↔ Vex Pro Side Bearing Gusset - OUT OF STOCK 1192014:1
- Mate:320: #8 1 in length standoff 93330A459:1 ↔ Vex Pro Side Bearing Gusset - OUT OF STOCK 1192014:1
- Mate:321: #8 1 in length standoff 93330A459:2 ↔ Vex Pro Side Bearing Gusset - OUT OF STOCK 1192014:2
- Mate:322: #8 1 in length standoff 93330A459:2 ↔ Vex Pro Side Bearing Gusset - OUT OF STOCK 1192014:1
- Mate:323: #8 1 in length standoff 93330A459:5 ↔ Vex Pro Side Bearing Gusset - OUT OF STOCK 1192014:2
- Mate:324: #8 1 in length standoff 93330A459:5 ↔ Vex Pro Side Bearing Gusset - OUT OF STOCK 1192014:1
- Mate:325: #8 1 in length standoff 93330A459:6 ↔ Vex Pro Side Bearing Gusset - OUT OF STOCK 1192014:2
- Mate:326: #8 1 in length standoff 93330A459:6 ↔ Vex Pro Side Bearing Gusset - OUT OF STOCK 1192014:1
- Mate:327: #8 1 in length standoff 93330A459:3 ↔ Vex Pro End Bearing Mount - IN STOCK 1192014:3
- Mate:328: #8 1 in length standoff 93330A459:3 ↔ Vex Pro End Bearing Mount - IN STOCK 1192014:3
- Mate:329: #8 1 in length standoff 93330A459:4 ↔ Vex Pro End Bearing Mount - IN STOCK 1192014:1
- Mate:330: #8 1 in length standoff 93330A459:4 ↔ Vex Pro End Bearing Mount - IN STOCK 1192014:3
- Mate:332: #8 1 in length standoff 93330A459:8 ↔ Vex Pro End Bearing Mount - IN STOCK 1192014:1
- Mate:333: #8 1 in length standoff 93330A459:8 ↔ Vex Pro End Bearing Mount - IN STOCK 1192014:3
- Mate:334: #8 1 in length standoff 93330A459:7 ↔ Vex Pro End Bearing Mount - IN STOCK 1192014:1
- Mate:335: #8 1 in length standoff 93330A459:7 ↔ Vex Pro End Bearing Mount - IN STOCK 1192014:3
- Mate:336: #8 1 in length standoff 93330A459:9 ↔ Vex Pro Side Bearing Gusset - OUT OF STOCK 1192014:4
- Mate:337: #8 1 in length standoff 93330A459:9 ↔ Vex Pro Side Bearing Gusset - OUT OF STOCK 1192014:3
- Mate:338: #8 1 in length standoff 93330A459:10 ↔ Vex Pro Side Bearing Gusset - OUT OF STOCK 1192014:3
- Mate:339: #8 1 in length standoff 93330A459:10 ↔ Vex Pro Side Bearing Gusset - OUT OF STOCK 1192014:3
- Mate:340: #8 1 in length standoff 93330A459:11 ↔ Vex Pro Side Bearing Gusset - OUT OF STOCK 1192014:3
- Mate:341: #8 1 in length standoff 93330A459:11 ↔ Vex Pro Side Bearing Gusset - OUT OF STOCK 1192014:4
- Mate:342: #8 1 in length standoff 93330A459:12 ↔ Vex Pro Side Bearing Gusset - OUT OF STOCK 1192014:3
- Mate:343: #8 1 in length standoff 93330A459:12 ↔ Vex Pro Side Bearing Gusset - OUT OF STOCK 1192014:3
- Mate:344: #8 1 in length standoff 93330A459:16 ↔ Vex Pro End Bearing Mount - IN STOCK 1192014:2
- Mate:345: #8 1 in length standoff 93330A459:16 ↔ Vex Pro End Bearing Mount - IN STOCK 1192014:4
- Mate:346: #8 1 in length standoff 93330A459:15 ↔ Vex Pro End Bearing Mount - IN STOCK 1192014:4
- Mate:347: #8 1 in length standoff 93330A459:15 ↔ Vex Pro End Bearing Mount - IN STOCK 1192014:2
- Mate:348: #8 1 in length standoff 93330A459:14 ↔ Vex Pro End Bearing Mount - IN STOCK 1192014:4
- Mate:349: #8 1 in length standoff 93330A459:14 ↔ Vex Pro End Bearing Mount - IN STOCK 1192014:4
- Mate:350: #8 1 in length standoff 93330A459:13 ↔ Vex Pro End Bearing Mount - IN STOCK 1192014:4
- Mate:351: #8 1 in length standoff 93330A459:13 ↔ Vex Pro End Bearing Mount - IN STOCK 1192014:2
- Mate:352: Vex Pro 1x1 rectangular tubing 12 in length:1 ↔ Ramp:2
- Mate:355: Vex Pro 1x1 rectangular tubing 12 in length:2 ↔ Ramp:1
- Mate:359: Vex Pro 1x1 rectangular tubing 7 in length:2 ↔ Ramp:2
- Mate:360: Vex Pro 1x1 rectangular tubing 7 in length:1 ↔ Ramp:1
- Mate:369: Vex Pro 1x1 rectangular tubing 9 in length:3 ↔ Vex Pro 1x1 rectangular tubing 6.125 in length:1
- Flush:66: Vex Pro 1x1 rectangular tubing 9 in length:3 ↔ Vex Pro 1x1 rectangular tubing 6.125 in length:1
- Mate:370: Vex Pro 1x1 rectangular tubing 6.125 in length:1 ↔ Vex Pro Corner Gusset - IN STOCK 1192014:21
- Flush:67: Vex Pro 1x1 rectangular tubing 25 in length:1 ↔ Vex Pro Corner Gusset - IN STOCK 1192014:21
- Flush:68: Vex Pro 1x1 rectangular tubing 6.125 in length:1 ↔ Vex Pro Corner Gusset - IN STOCK 1192014:21
- Mate:375: Vex Pro T gusset - OUT OF STOCK 1192014:1 ↔ Vex Pro 1x1 rectangular tubing 12 in length:2
- Flush:69: Vex Pro T gusset - OUT OF STOCK 1192014:1 ↔ Vex Pro 1x1 rectangular tubing 12 in length:2
- Flush:70: Vex Pro T gusset - OUT OF STOCK 1192014:1 ↔ Vex Pro 1x1 rectangular tubing 13 in length:1
- Mate:376: Vex Pro T gusset - OUT OF STOCK 1192014:2 ↔ Vex Pro 1x1 rectangular tubing 12 in length:1
- Flush:71: Vex Pro T gusset - OUT OF STOCK 1192014:2 ↔ Vex Pro 1x1 rectangular tubing 12 in length:1
- Flush:72: Vex Pro T gusset - OUT OF STOCK 1192014:2 ↔ Vex Pro 1x1 rectangular tubing 13 in length:1
- Mate:377: D-9969:1 ↔ 176-DP(D-229)(F,D-231-1):1
- Mate:378: Vex Pro 1x1 rectangular tubing 12 in length:2 ↔ #8 0.250 in length spacer 92510A462:2
- Mate:379: #8 0.250 in length spacer 92510A462:2 ↔ Ramp:1
- Mate:380: Vex Pro 1x1 rectangular tubing 12 in length:1 ↔ #8 0.250 in length spacer 92510A462:1
- Mate:381: Vex Pro 1x1 rectangular tubing 12 in length:1 ↔ #8 0.250 in length spacer 92510A462:1
- Mate:382: #8 0.250 in length spacer 92510A462:1 ↔ Ramp:2
- Mate:383: #8 0.250 in length spacer 92510A462:2 ↔ Ramp:1
- Mate:384: #8 0.625 in length spacer 92510A466:1 ↔ Ramp:2
- Mate:385: Vex Pro 1x1 rectangular tubing 7 in length:2 ↔ #8 0.625 in length spacer 92510A466:1
- Mate:386: #8 0.625 in length spacer 92510A466:2 ↔ Ramp:1
- Mate:387: Vex Pro 1x1 rectangular tubing 7 in length:1 ↔ #8 0.625 in length spacer 92510A466:2
- Mate:388: Vex Pro T gusset - OUT OF STOCK 1192014:3 ↔ Vex Pro 1x1 rectangular tubing 13 in length:1
- Flush:73: Vex Pro T gusset - OUT OF STOCK 1192014:3 ↔ Vex Pro 1x1 rectangular tubing 13 in length:1
- Flush:74: Vex Pro T gusset - OUT OF STOCK 1192014:3 ↔ Vex Pro 1x1 rectangular tubing 25 in length:1
- Mate:389: Vex Pro 1x1 rectangular tubing 12 in length:2 ↔ Vex Pro Corner Gusset - IN STOCK 1192014:2
- Flush:75: Vex Pro 1x1 rectangular tubing 12 in length:2 ↔ Vex Pro Corner Gusset - IN STOCK 1192014:2
- Flush:76: Vex Pro 1x1 rectangular tubing 12 in length:2 ↔ Vex Pro Corner Gusset - IN STOCK 1192014:2
- Mate:390: Vex Pro 1x1 rectangular tubing 12 in length:1 ↔ Vex Pro Corner Gusset - IN STOCK 1192014:4
- Flush:77: Vex Pro 1x1 rectangular tubing 12 in length:1 ↔ Vex Pro Corner Gusset - IN STOCK 1192014:4
- Flush:78: Vex Pro 1x1 rectangular tubing 12 in length:1 ↔ Vex Pro Corner Gusset - IN STOCK 1192014:4
- Mate:391: Vex Pro 1x1 rectangular tubing 7 in length:2 ↔ Vex Pro Corner Gusset - IN STOCK 1192014:6
- Flush:79: Vex Pro 1x1 rectangular tubing 7 in length:2 ↔ Vex Pro Corner Gusset - IN STOCK 1192014:6
- Flush:80: Vex Pro 1x1 rectangular tubing 7 in length:2 ↔ Vex Pro Corner Gusset - IN STOCK 1192014:6
- Mate:392: Vex Pro 1x1 rectangular tubing 7 in length:1 ↔ Vex Pro Corner Gusset - IN STOCK 1192014:8
- Flush:81: Vex Pro 1x1 rectangular tubing 7 in length:1 ↔ Vex Pro Corner Gusset - IN STOCK 1192014:8
- Flush:82: Vex Pro 1x1 rectangular tubing 7 in length:1 ↔ Vex Pro Corner Gusset - IN STOCK 1192014:8
- Mate:397: Bearing ID 0.500 Hex OD 1.125:7 ↔ Spacer (0.630 in ID 1 in OD) aluminum:2
- Mate:398: Spacer (0.630 in ID 1 in OD) aluminum:2 ↔ Hex Shaft Collar 1-2 in (7552K500):5
- Mate:399: Spacer (0.630 in ID 1 in OD) aluminum:1 ↔ Hex Shaft Collar 1-2 in (7552K500):3
- Mate:400: Spacer (0.630 in ID 1 in OD) aluminum:1 ↔ Hex Shaft Collar 1-2 in (7552K500):3
- Mate:403 (12.7 mm): Vex Pro 1x1 rectangular tubing 12 in length:1 ↔ Pneumatics_Clippard_AVT-32-32:1
- Tangent:2 (-63.5 mm): Pneumatics_Clippard_AVT-32-32:1 ↔ Vex Pro 1x1 rectangular tubing 13 in length:1
- Flush:87: Pneumatics_Clippard_AVT-32-32:1 ↔ Pneumatics_Clippard_AVT-32-32:2
- Mate:404: Pneumatics Board:1 ↔ Vex Pro 1x1 rectangular tubing 13 in length:1
- Mate:405: Vex Pro 1x1 rectangular tubing 12 in length:1 ↔ Pneumatics Board:1
- Flush:89: Pneumatics Board:1 ↔ Vex Pro 1x1 rectangular tubing 13 in length:1
- Mate:406: Manifold:1 ↔ Pneumatics Board:1
- Mate:408: pneumatic thing 1:1 ↔ Pneumatics Board:1
- Mate:409: CS_WirelessBridge_DAP1522:1 ↔ Pneumatics Board:1
- Mate:410: CS_Converter_CLL25-24S05:1 ↔ Pneumatics Board:1
- Flush:90 (12.7 mm): CS_WirelessBridge_DAP1522:1 ↔ Pneumatics Board:1
- Flush:91 (12.7 mm): CS_WirelessBridge_DAP1522:1 ↔ Pneumatics Board:1
- Flush:92 (12.7 mm): pneumatic thing 1:1 ↔ Pneumatics Board:1
- Flush:93 (25.4 mm): pneumatic thing 1:1 ↔ Pneumatics Board:1
- Tangent:7: Pneumatics_Clippard_AVT-32-32:2 ↔ Pneumatics Board:1
- Tangent:8: Pneumatics_Clippard_AVT-32-16:1 ↔ Pneumatics Board:1
- Tangent:9: Pneumatics_Clippard_AVT-32-32:1 ↔ Pneumatics Board:1
- Tangent:10: Pneumatics_Clippard_AVT-32-16:2 ↔ Pneumatics Board:1
- Flush:94: Pneumatics_Clippard_AVT-32-16:1 ↔ Pneumatics_Clippard_AVT-32-16:2
- Mate:413: Pneumatics Board:1 ↔ pneumatics thing 2:2
- Tangent:11: Pneumatics_Clippard_AVT-32-16:1 ↔ Pneumatics_Clippard_AVT-32-16:2
- Flush:97 (50.8 mm): Manifold:1 ↔ Pneumatics Board:1
- Mate:414: CS_Converter_CLL25-24S05:1 ↔ Pneumatics Board:1
- Mate:415: CS_Converter_CLL25-24S05:1 ↔ Pneumatics Board:1
- Flush:98 (59.69 mm): Manifold:1 ↔ Pneumatics Board:1
- Flush:99 (22.225 mm): Pneumatics Board:1 ↔ pneumatics thing 2:2
- Flush:100 (5.08 mm): Pneumatics Board:1 ↔ pneumatics thing 2:2
- Tangent:12: Pneumatics_Clippard_AVT-32-16:1 ↔ Pneumatics_Clippard_AVT-32-32:1
- Tangent:13: Pneumatics_Clippard_AVT-32-16:2 ↔ Pneumatics_Clippard_AVT-32-32:2
- Flush:101 (63.5 mm): Pneumatics_Clippard_AVT-32-16:2 ↔ Pneumatics_Clippard_AVT-32-32:2
- Mate:416: Vex Pro 1x1 rectangular tubing 25 in length:1 ↔ FO-022:1
- Mate:417: Vex Pro 1x1 rectangular tubing 25 in length:1 ↔ FO-022:1
- Mate:418: Pneumatics Board:1 ↔ Aluminum Angle 2:1
- Flush:102: Pneumatics Board:1 ↔ Aluminum Angle 2:1
- Mate:419: Pneumatics Board:1 ↔ Aluminum Angle 2:1
- Mate:420: Pneumatics Board:1 ↔ Aluminum Angle 2:2
- Flush:103: Pneumatics Board:1 ↔ Aluminum Angle 2:2
- Mate:421: Pneumatics Board:1 ↔ Aluminum Angle 2:2
- Flush:104: Pneumatics Board:1 ↔ Aluminum Angle 1 Left:1
- Mate:422: Pneumatics Board:1 ↔ Aluminum Angle 1 Left:1
- Mate:423: Pneumatics Board:1 ↔ Aluminum Angle 1 Left:1
- Mate:424: Pneumatics Board:1 ↔ Aluminum Angle 1 Right:1
- Mate:425: Pneumatics Board:1 ↔ Aluminum Angle 1 Right:1
- Flush:105: Pneumatics Board:1 ↔ Aluminum Angle 1 Right:1
- Mate:426: Pneumatics Board:1 ↔ Aluminum Angle 3 Left:1
- Flush:106: Pneumatics Board:1 ↔ Aluminum Angle 3 Left:1
- Mate:427: Aluminum Angle 2:2 ↔ Aluminum Angle 3 Left:1
- Mate:428: Pneumatics Board:1 ↔ Aluminum Angle 3 Right:1
- Mate:429: Aluminum Angle 2:1 ↔ Aluminum Angle 3 Right:1
- Flush:107: Pneumatics Board:1 ↔ Aluminum Angle 3 Right:1
- Mate:430: Aluminum Plate (0.125):2 ↔ Vex Pro 1x1 rectangular tubing 7 in length:2
- Mate:431: Aluminum Plate (0.125):2 ↔ Vex Pro 1x1 rectangular tubing 7 in length:2
- Mate:432: Aluminum Plate (0.125):2 ↔ 176-DP(D-229)(F,D-231-1):1
- Mate:433: Aluminum Plate (0.125):2 ↔ 176-DP(D-229)(F,D-231-1):1
- Mate:434: Aluminum Plate (0.125):1 ↔ Vex Pro 1x1 rectangular tubing 7 in length:1
- Mate:435: Aluminum Plate (0.125):1 ↔ Vex Pro 1x1 rectangular tubing 7 in length:1
- Mate:436: Aluminum Plate (0.125):1 ↔ 176-DP(D-229)(F,D-231-1):2
- Mate:437: Aluminum Plate (0.125):1 ↔ 176-DP(D-229)(F,D-231-1):2
